# Autodesk Inventor assembly: 2016 new frame
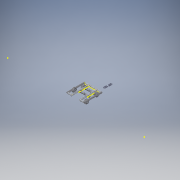
[picture p0: Inventor's stored thumbnail of the model, 180x180]
Saved by Autodesk Inventor 2017 (Build 210142000, 142)
## iProperties
Created: 2016-12-13
Part Number: 2016 new frame
Document SubType Name: Assembly
Designer: Aditya
Author: Aditya
## Documents named in this file (14)
- C:\Users\Aditya\Documents\GitHub\RobotuxCAD\Team Robotux 15-16 Robot Cad Assets\2016 new frame.iam
- C:\Users\Aditya\Documents\GitHub\RobotuxCAD\Team Robotux 15-16 Robot Cad Assets\Andy Mark Parts\15in 1in alu ext.ipt
- C:\Users\Aditya\Documents\GitHub\RobotuxCAD\Team Robotux 15-16 Robot Cad Assets\Andy Mark Parts\4in long 1 in extrusion.ipt
- C:\Users\Aditya\Documents\GitHub\RobotuxCAD\Team Robotux 15-16 Robot Cad Assets\Andy Mark Parts\REV-21-1000.ipt
- C:\Users\Aditya\Documents\GitHub\RobotuxCAD\Team Robotux 15-16 Robot Cad Assets\Andy Mark Parts\4HD Mecanum Left.ipt
- C:\Users\Aditya\Documents\GitHub\RobotuxCAD\Team Robotux 15-16 Robot Cad Assets\Andy Mark Parts\4HD Mecanum Right.ipt
- C:\Users\Aditya\Documents\GitHub\RobotuxCAD\Team Robotux 15-16 Robot Cad Assets\Andy Mark Parts\1in corner bracket for extrusions.ipt
- C:\Users\Aditya\Documents\GitHub\RobotuxCAD\Team Robotux 15-16 Robot Cad Assets\Andy Mark Parts\1in corner bracket for extrusions cut.ipt
- C:\Users\Aditya\Documents\GitHub\RobotuxCAD\Team Robotux 15-16 Robot Cad Assets\Andy Mark Parts\am-2609a+FTC+Conversion+Plate+REV+2.ipt
- C:\Users\Aditya\Documents\GitHub\RobotuxCAD\Team Robotux 15-16 Robot Cad Assets\Andy Mark Parts\am-3052_72in_C_Channel.ipt
- C:\Users\Aditya\Documents\GitHub\RobotuxCAD\Team Robotux 15-16 Robot Cad Assets\Drive Motor Plate.ipt
- C:\Users\Aditya\Documents\GitHub\RobotuxCAD\Team Robotux 15-16 Robot Cad Assets\Tetrix Parts\tetrix_739089_2012.ipt
- C:\Users\Aditya\Documents\GitHub\RobotuxCAD\Team Robotux 15-16 Robot Cad Assets\Andy Mark Parts\am-2964NeveRest.ipt
- C:\Users\Aditya\Documents\GitHub\RobotuxCAD\Team Robotux 15-16 Robot Cad Assets\Tetrix Parts\tetrix_739079_collar_2012.ipt
## Components (45 placed, 13 different names)
1. 15in 1in alu ext:1 — Mate:1, Flush:1, Flush:2, Mate:2, Flush:3, Flush:4, Flush:22, Flush:27, Mate:54, Flush:40, Mate:55, Flush:42
2. 15in 1in alu ext:2 — Mate:4, Flush:7, Flush:8, Mate:16, Flush:32, Mate:49, Flush:37, Flush:43, Mate:67, Flush:47
3. 15in 1in alu ext:3 — Mate:6, Flush:11, Flush:12, Mate:15, Flush:29, Mate:51, Flush:38, Flush:41, Mate:66, Flush:46
4. 4in long 1 in extrusion:1 — Mate:3, Flush:5, Flush:6, Mate:4, Flush:7, Flush:8, Mate:10, Flush:19, Flush:31
5. 4in long 1 in extrusion:2 — Mate:5, Flush:9, Flush:10, Mate:6, Flush:11, Flush:12, Mate:9, Flush:18, Flush:30
6. REV-21-1000:1 — Mate:2, Flush:3, Flush:4, Mate:3, Flush:5, Flush:6, Flush:20, Mate:14, Flush:28
7. REV-21-1000:2 — Mate:1, Flush:1, Flush:2, Mate:5, Flush:9, Flush:10, Flush:17, Mate:11, Flush:21
8. 4HD Mecanum Left:1 — Mate:25, Mate:26, Mate:27, Mate:28, Mate:29, Mate:30, Mate:81
9. 4HD Mecanum Left:2 — Mate:19, Mate:20, Mate:21, Mate:22, Mate:23, Mate:24, Mate:53
10. 4HD Mecanum Right:1 — Mate:31, Mate:32, Mate:33, Mate:34, Mate:35, Mate:36
11. 4HD Mecanum Right:2 — Mate:37, Mate:38, Mate:39, Mate:40, Mate:41, Mate:42, Mate:57
12. 1in corner bracket for extrusions:1 — Mate:11, Flush:21, Flush:22
13. 1in corner bracket for extrusions:3 — Mate:14, Flush:27, Flush:28
14. 1in corner bracket for extrusions:11 — Mate:9, Flush:17, Flush:18
15. 1in corner bracket for extrusions:12 — Mate:10, Flush:19, Flush:20
16. 1in corner bracket for extrusions cut:1 — Mate:16, Flush:31, Flush:32
17. 1in corner bracket for extrusions cut:2 — Mate:15, Flush:29, Flush:30
18. 1in corner bracket for extrusions:13 — Mate:55, Flush:42, Flush:43
19. 1in corner bracket for extrusions:14 — Mate:54, Flush:40, Flush:41
20. am-2609a+FTC+Conversion+Plate+REV+2:1 — Mate:28, Mate:29, Mate:30
21. am-2609a+FTC+Conversion+Plate+REV+2:2 — Mate:22, Mate:23, Mate:24, Mate:77
22. am-2609a+FTC+Conversion+Plate+REV+2:3 — Mate:25, Mate:26, Mate:27, Mate:80, Mate:82
23. am-2609a+FTC+Conversion+Plate+REV+2:4 — Mate:40, Mate:41, Mate:42, Mate:72
24. am-2609a+FTC+Conversion+Plate+REV+2:5 — Mate:37, Mate:38, Mate:39, Mate:74
25. am-2609a+FTC+Conversion+Plate+REV+2:6 — Mate:34, Mate:35, Mate:36
26. am-2609a+FTC+Conversion+Plate+REV+2:7 — Mate:31, Mate:32, Mate:33, Mate:78, Mate:79
27. am-2609a+FTC+Conversion+Plate+REV+2:8 — Mate:19, Mate:20, Mate:21, Mate:75
28. am-3052_72in_C_Channel:1
29. Drive Motor Plate:1 — Mate:43, Mate:44, Mate:45, Mate:49, Flush:37
30. Drive Motor Plate:2 — Mate:46, Mate:47, Mate:48, Mate:51, Flush:38
31. tetrix_739089_2012:1 — Mate:46, Mate:47, Mate:48, Mate:52, Flush:39
32. tetrix_739089_2012:2 — Mate:43, Mate:44, Mate:45, Flush:44, Mate:56
33. am-2964NeveRest:1 — Flush:44, Mate:56, Mate:57, Flush:45, Mate:70, Mate:73
34. am-2964NeveRest:2 — Mate:52, Mate:53, Flush:39, Flush:45, Mate:70, Mate:76
35. am-2964NeveRest:3 — Mate:68, Flush:48, Flush:51, Mate:71
36. am-2964NeveRest:4 — Mate:69, Flush:49, Flush:50, Flush:51, Mate:71
37. Drive Motor Plate:3 — Mate:62, Mate:63, Mate:64, Mate:65, Mate:66, Flush:46
38. Drive Motor Plate:4 — Mate:58, Mate:59, Mate:60, Mate:61, Mate:67, Flush:47
39. tetrix_739089_2012:3 — Mate:58, Mate:59, Mate:60, Mate:61, Mate:69, Flush:49, Flush:50
40. tetrix_739089_2012:4 — Mate:62, Mate:63, Mate:64, Mate:65, Mate:68, Flush:48
41. am-3052_72in_C_Channel:2
42. tetrix_739079_collar_2012:1 — Mate:78, Mate:79
43. tetrix_739079_collar_2012:2 — Mate:80, Mate:81, Mate:82
44. tetrix_739079_collar_2012:3 — Mate:75, Mate:76, Mate:77
45. tetrix_739079_collar_2012:4 — Mate:72, Mate:73, Mate:74
## Relationships (114: Mate 75, Flush 39)
- Mate:1: 15in 1in alu ext:1 ↔ REV-21-1000:2
- Flush:1: 15in 1in alu ext:1 ↔ REV-21-1000:2
- Flush:2: 15in 1in alu ext:1 ↔ REV-21-1000:2
- Mate:2: 15in 1in alu ext:1 ↔ REV-21-1000:1
- Flush:3: 15in 1in alu ext:1 ↔ REV-21-1000:1
- Flush:4: 15in 1in alu ext:1 ↔ REV-21-1000:1
- Mate:3: 4in long 1 in extrusion:1 ↔ REV-21-1000:1
- Flush:5: 4in long 1 in extrusion:1 ↔ REV-21-1000:1
- Flush:6: 4in long 1 in extrusion:1 ↔ REV-21-1000:1
- Mate:4: 15in 1in alu ext:2 ↔ 4in long 1 in extrusion:1
- Flush:7: 15in 1in alu ext:2 ↔ 4in long 1 in extrusion:1
- Flush:8: 15in 1in alu ext:2 ↔ 4in long 1 in extrusion:1
- Mate:5: 4in long 1 in extrusion:2 ↔ REV-21-1000:2
- Flush:9: 4in long 1 in extrusion:2 ↔ REV-21-1000:2
- Flush:10: 4in long 1 in extrusion:2 ↔ REV-21-1000:2
- Mate:6: 15in 1in alu ext:3 ↔ 4in long 1 in extrusion:2
- Flush:11: 15in 1in alu ext:3 ↔ 4in long 1 in extrusion:2
- Flush:12: 15in 1in alu ext:3 ↔ 4in long 1 in extrusion:2
- Mate:9: 4in long 1 in extrusion:2 ↔ 1in corner bracket for extrusions:11
- Flush:17: REV-21-1000:2 ↔ 1in corner bracket for extrusions:11
- Flush:18: 4in long 1 in extrusion:2 ↔ 1in corner bracket for extrusions:11
- Mate:10: 4in long 1 in extrusion:1 ↔ 1in corner bracket for extrusions:12
- Flush:19: 4in long 1 in extrusion:1 ↔ 1in corner bracket for extrusions:12
- Flush:20: REV-21-1000:1 ↔ 1in corner bracket for extrusions:12
- Mate:11: REV-21-1000:2 ↔ 1in corner bracket for extrusions:1
- Flush:21: REV-21-1000:2 ↔ 1in corner bracket for extrusions:1
- Flush:22: 15in 1in alu ext:1 ↔ 1in corner bracket for extrusions:1
- Mate:14: REV-21-1000:1 ↔ 1in corner bracket for extrusions:3
- Flush:27: 15in 1in alu ext:1 ↔ 1in corner bracket for extrusions:3
- Flush:28: REV-21-1000:1 ↔ 1in corner bracket for extrusions:3
- Mate:15: 15in 1in alu ext:3 ↔ 1in corner bracket for extrusions cut:2
- Flush:29: 15in 1in alu ext:3 ↔ 1in corner bracket for extrusions cut:2
- Flush:30: 4in long 1 in extrusion:2 ↔ 1in corner bracket for extrusions cut:2
- Mate:16: 15in 1in alu ext:2 ↔ 1in corner bracket for extrusions cut:1
- Flush:31: 4in long 1 in extrusion:1 ↔ 1in corner bracket for extrusions cut:1
- Flush:32: 15in 1in alu ext:2 ↔ 1in corner bracket for extrusions cut:1
- Mate:19: 4HD Mecanum Left:2 ↔ am-2609a+FTC+Conversion+Plate+REV+2:8
- Mate:20: 4HD Mecanum Left:2 ↔ am-2609a+FTC+Conversion+Plate+REV+2:8
- Mate:21: 4HD Mecanum Left:2 ↔ am-2609a+FTC+Conversion+Plate+REV+2:8
- Mate:22: 4HD Mecanum Left:2 ↔ am-2609a+FTC+Conversion+Plate+REV+2:2
- Mate:23: 4HD Mecanum Left:2 ↔ am-2609a+FTC+Conversion+Plate+REV+2:2
- Mate:24: 4HD Mecanum Left:2 ↔ am-2609a+FTC+Conversion+Plate+REV+2:2
- Mate:25: 4HD Mecanum Left:1 ↔ am-2609a+FTC+Conversion+Plate+REV+2:3
- Mate:26: 4HD Mecanum Left:1 ↔ am-2609a+FTC+Conversion+Plate+REV+2:3
- Mate:27: 4HD Mecanum Left:1 ↔ am-2609a+FTC+Conversion+Plate+REV+2:3
- Mate:28: 4HD Mecanum Left:1 ↔ am-2609a+FTC+Conversion+Plate+REV+2:1
- Mate:29: 4HD Mecanum Left:1 ↔ am-2609a+FTC+Conversion+Plate+REV+2:1
- Mate:30: 4HD Mecanum Left:1 ↔ am-2609a+FTC+Conversion+Plate+REV+2:1
- Mate:31: 4HD Mecanum Right:1 ↔ am-2609a+FTC+Conversion+Plate+REV+2:7
- Mate:32: 4HD Mecanum Right:1 ↔ am-2609a+FTC+Conversion+Plate+REV+2:7
- Mate:33: 4HD Mecanum Right:1 ↔ am-2609a+FTC+Conversion+Plate+REV+2:7
- Mate:34: 4HD Mecanum Right:1 ↔ am-2609a+FTC+Conversion+Plate+REV+2:6
- Mate:35: 4HD Mecanum Right:1 ↔ am-2609a+FTC+Conversion+Plate+REV+2:6
- Mate:36: 4HD Mecanum Right:1 ↔ am-2609a+FTC+Conversion+Plate+REV+2:6
- Mate:37: 4HD Mecanum Right:2 ↔ am-2609a+FTC+Conversion+Plate+REV+2:5
- Mate:38: 4HD Mecanum Right:2 ↔ am-2609a+FTC+Conversion+Plate+REV+2:5
- Mate:39: 4HD Mecanum Right:2 ↔ am-2609a+FTC+Conversion+Plate+REV+2:5
- Mate:40: 4HD Mecanum Right:2 ↔ am-2609a+FTC+Conversion+Plate+REV+2:4
- Mate:41: 4HD Mecanum Right:2 ↔ am-2609a+FTC+Conversion+Plate+REV+2:4
- Mate:42: 4HD Mecanum Right:2 ↔ am-2609a+FTC+Conversion+Plate+REV+2:4
- Mate:43: Drive Motor Plate:1 ↔ tetrix_739089_2012:2
- Mate:44: Drive Motor Plate:1 ↔ tetrix_739089_2012:2
- Mate:45: Drive Motor Plate:1 ↔ tetrix_739089_2012:2
- Mate:46: Drive Motor Plate:2 ↔ tetrix_739089_2012:1
- Mate:47: Drive Motor Plate:2 ↔ tetrix_739089_2012:1
- Mate:48: Drive Motor Plate:2 ↔ tetrix_739089_2012:1
- Mate:49: 15in 1in alu ext:2 ↔ Drive Motor Plate:1
- Flush:37: 15in 1in alu ext:2 ↔ Drive Motor Plate:1
- Mate:51: 15in 1in alu ext:3 ↔ Drive Motor Plate:2
- Flush:38: 15in 1in alu ext:3 ↔ Drive Motor Plate:2
- Mate:52: tetrix_739089_2012:1 ↔ am-2964NeveRest:2
- Mate:53: 4HD Mecanum Left:2 ↔ am-2964NeveRest:2
- Flush:39: tetrix_739089_2012:1 ↔ am-2964NeveRest:2
- Mate:54: 15in 1in alu ext:1 ↔ 1in corner bracket for extrusions:14
- Flush:40: 15in 1in alu ext:1 ↔ 1in corner bracket for extrusions:14
- Flush:41: 15in 1in alu ext:3 ↔ 1in corner bracket for extrusions:14
- Mate:55: 15in 1in alu ext:1 ↔ 1in corner bracket for extrusions:13
- Flush:42: 15in 1in alu ext:1 ↔ 1in corner bracket for extrusions:13
- Flush:43: 15in 1in alu ext:2 ↔ 1in corner bracket for extrusions:13
- Flush:44: tetrix_739089_2012:2 ↔ am-2964NeveRest:1
- Mate:56: tetrix_739089_2012:2 ↔ am-2964NeveRest:1
- Mate:57: 4HD Mecanum Right:2 ↔ am-2964NeveRest:1
- Flush:45: am-2964NeveRest:1 ↔ am-2964NeveRest:2
- Mate:58: Drive Motor Plate:4 ↔ tetrix_739089_2012:3
- Mate:59: Drive Motor Plate:4 ↔ tetrix_739089_2012:3
- Mate:60: Drive Motor Plate:4 ↔ tetrix_739089_2012:3
- Mate:61: Drive Motor Plate:4 ↔ tetrix_739089_2012:3
- Mate:62: Drive Motor Plate:3 ↔ tetrix_739089_2012:4
- Mate:63: Drive Motor Plate:3 ↔ tetrix_739089_2012:4
- Mate:64: Drive Motor Plate:3 ↔ tetrix_739089_2012:4
- Mate:65: Drive Motor Plate:3 ↔ tetrix_739089_2012:4
- Mate:66: 15in 1in alu ext:3 ↔ Drive Motor Plate:3
- Flush:46: 15in 1in alu ext:3 ↔ Drive Motor Plate:3
- Mate:67: 15in 1in alu ext:2 ↔ Drive Motor Plate:4
- Flush:47: 15in 1in alu ext:2 ↔ Drive Motor Plate:4
- Mate:68: am-2964NeveRest:3 ↔ tetrix_739089_2012:4
- Mate:69: am-2964NeveRest:4 ↔ tetrix_739089_2012:3
- Flush:48: am-2964NeveRest:3 ↔ tetrix_739089_2012:4
- Flush:49: am-2964NeveRest:4 ↔ tetrix_739089_2012:3
- Flush:50: am-2964NeveRest:4 ↔ tetrix_739089_2012:3
- Flush:51: am-2964NeveRest:3 ↔ am-2964NeveRest:4
- Mate:70: am-2964NeveRest:1 ↔ am-2964NeveRest:2
- Mate:71: am-2964NeveRest:3 ↔ am-2964NeveRest:4
- Mate:72: am-2609a+FTC+Conversion+Plate+REV+2:4 ↔ tetrix_739079_collar_2012:4
- Mate:73: am-2964NeveRest:1 ↔ tetrix_739079_collar_2012:4
- Mate:74: am-2609a+FTC+Conversion+Plate+REV+2:5 ↔ tetrix_739079_collar_2012:4
- Mate:75: am-2609a+FTC+Conversion+Plate+REV+2:8 ↔ tetrix_739079_collar_2012:3
- Mate:76: am-2964NeveRest:2 ↔ tetrix_739079_collar_2012:3
- Mate:77: am-2609a+FTC+Conversion+Plate+REV+2:2 ↔ tetrix_739079_collar_2012:3
- Mate:78: am-2609a+FTC+Conversion+Plate+REV+2:7 ↔ tetrix_739079_collar_2012:1
- Mate:79: am-2609a+FTC+Conversion+Plate+REV+2:7 ↔ tetrix_739079_collar_2012:1
- Mate:80: am-2609a+FTC+Conversion+Plate+REV+2:3 ↔ tetrix_739079_collar_2012:2
- Mate:81: 4HD Mecanum Left:1 ↔ tetrix_739079_collar_2012:2
- Mate:82: am-2609a+FTC+Conversion+Plate+REV+2:3 ↔ tetrix_739079_collar_2012:2
